# Autodesk Inventor assembly: camera_jig
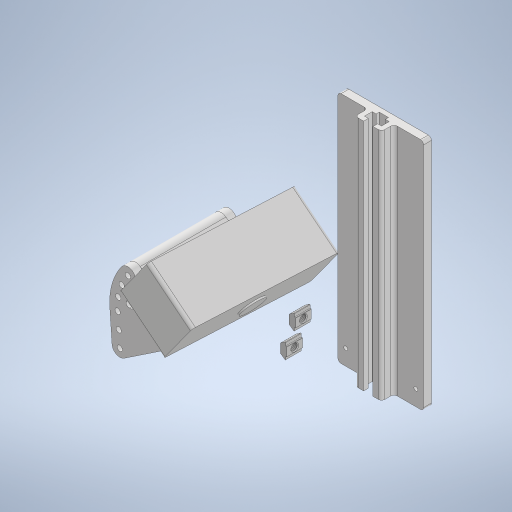
[picture p0: Inventor's stored thumbnail of the model, 512x512]
Saved by Autodesk Inventor 2024.3 (Build 283343010, 343A)
## iProperties
Created: 2025-07-19
Part Number: camera_jig
Document SubType Name: Assembly
Designer: hikou
Author: hikou
## Documents named in this file (8)
- C:\Users\hikou\OneDrive\ドキュメント\Inventor\harvesting_robot\camera_jig\camera_jig.iam
- C:\Users\hikou\OneDrive\ドキュメント\Inventor\harvesting_robot\camera_jig\camera_connect_part.ipt
- C:\Users\hikou\OneDrive\ドキュメント\Inventor\harvesting_robot\camera_jig\side_part.ipt
- C:\Users\hikou\OneDrive\ドキュメント\Inventor\harvesting_robot\camera_jig\slide_part.ipt
- C:\Users\hikou\OneDrive\ドキュメント\Inventor\harvesting_robot\camera_jig\center_part.ipt
- C:\Users\hikou\OneDrive\ドキュメント\Inventor\harvesting_robot\camera_jig\CBE5-15.ipt
- C:\Users\hikou\OneDrive\ドキュメント\Inventor\harvesting_robot\camera_jig\AIS2024\HNTTSS5-5.ipt
- C:\Users\hikou\OneDrive\ドキュメント\Inventor\harvesting_robot\camera_jig\zed_x_mini.ipt
## Components (10 placed, 7 different names)
1. camera_connect_part:1 — 回転:1, 挿入:11
2. side_part:1 — 挿入:6, 回転:1, 挿入:9
3. side_part:2 — 挿入:5, 挿入:10
4. slide_part:1
5. center_part:1 — 挿入:5, 挿入:6, 挿入:7, 挿入:8, 挿入:9, 挿入:10
6. CBE5-15:1 — 挿入:8
7. CBE5-15:2 — 挿入:7
8. HNTTSS5-5:1
9. HNTTSS5-5:2
10. zed_x_mini:1 — 挿入:11
## Relationships (8: Insert 7, RevoluteJoint 1)
- 挿入:5 [Insert]: side_part:2 ↔ center_part:1
- 挿入:6 [Insert]: side_part:1 ↔ center_part:1
- 挿入:7 [Insert]: center_part:1 ↔ CBE5-15:2
- 挿入:8 [Insert]: center_part:1 ↔ CBE5-15:1
- 回転:1 [RevoluteJoint]: camera_connect_part:1 ↔ side_part:1
- 挿入:9 [Insert]: side_part:1 ↔ center_part:1
- 挿入:10 [Insert]: side_part:2 ↔ center_part:1
- 挿入:11 [Insert]: camera_connect_part:1 ↔ zed_x_mini:1
